# Autodesk Inventor assembly: Full Keyboard
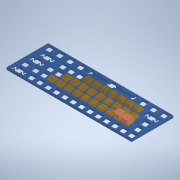
[picture p0: Inventor's stored thumbnail of the model, 180x180]
Saved by Autodesk Inventor 2022 (Build 260153000, 153)
## iProperties
Created: 2022-03-01
Part Number: Full Keyboard
Document SubType Name: Assembly
Designer: Nathan Griffith
Author: Nathan Griffith
## Documents named in this file (5)
- C:\Users\Nathan Griffith\Documents\Inventor\Eric's Keyboard\Full Keyboard.iam
- C:\Users\Nathan Griffith\Documents\Inventor\Eric's Keyboard\plate.ipt
- C:\Users\Nathan Griffith\Documents\Inventor\Eric's Keyboard\cherry mx.ipt
- C:\Users\Nathan Griffith\Documents\Inventor\Eric's Keyboard\Keycap a-z\KeycapQ.ipt
- C:\Users\Nathan Griffith\Documents\Inventor\Eric's Keyboard\Keycap a-z\KeycapW.ipt
## Components (29 placed, 4 different names)
1. plate:1 — Mate:1, Mate:2, Mate:3, Mate:4, Mate:5
2. KeycapQ:1 — Mate:6
3. KeycapW:1 — Mate:7
4. cherry mx:1 — Mate:1, Mate:2, Mate:6
5. cherry mx:2 — Mate:7
6. cherry mx:3
7. cherry mx:4
8. cherry mx:5
9. cherry mx:6
10. cherry mx:7
11. cherry mx:8
12. cherry mx:9
13. cherry mx:10
14. cherry mx:11 — Mate:3, Mate:4
15. cherry mx:12
16. cherry mx:13
17. cherry mx:14
18. cherry mx:15
19. cherry mx:16
20. cherry mx:17
21. cherry mx:18
22. cherry mx:19
23. cherry mx:20 — Mate:5
24. cherry mx:21
25. cherry mx:22
26. cherry mx:23
27. cherry mx:24
28. cherry mx:25
29. cherry mx:26
## Component patterns: (10 elements, first: cherry mx:1), (9 elements, first: cherry mx:11), (7 elements, first: cherry mx:20)
## Relationships (7: Mate 7)
- Mate:1: plate:1 ↔ cherry mx:1
- Mate:2: plate:1 ↔ cherry mx:1
- Mate:3: plate:1 ↔ cherry mx:11
- Mate:4: plate:1 ↔ cherry mx:11
- Mate:5: plate:1 ↔ cherry mx:20
- Mate:6: KeycapQ:1 ↔ cherry mx:1
- Mate:7: KeycapW:1 ↔ cherry mx:2
